# Autodesk Inventor assembly: MIR_HbHand
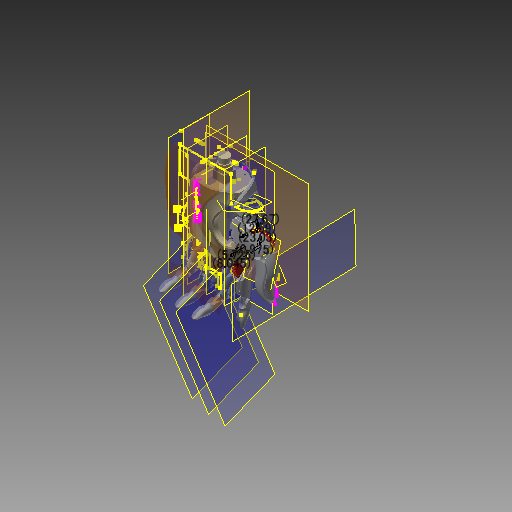
[picture p0: Inventor's stored thumbnail of the model, 512x512]
Saved by Autodesk Inventor 2017 (Build 210142000, 142)
## iProperties
Part Number: MIR_HbHand
Material: 一般
Document SubType Name: Assembly
Designer: sktom
Author: sktom
## Documents named in this file (23)
- D:\OneDrive\CAD\MAJ\hackberry\HACKberry-hardware\3D_69%inlength\Inventor\HbHandForChild\MIR_HbHand.iam
- D:\OneDrive\CAD\MAJ\hackberry\HACKberry-hardware\3D_69%inlength\Inventor\HbHandForChild\MIR_HbPalmBase03ForChild.ipt
- D:\OneDrive\CAD\MAJ\hackberry\HACKberry-hardware\3D_69%inlength\Inventor\HbHandForChild\MIR_bearing_683.ipt
- D:\OneDrive\CAD\MAJ\hackberry\HACKberry-hardware\3D_69%inlength\Inventor\HbHandForChild\HbthumbU02ForChild\MIR_HbthumbU02ForChild.iam
- D:\OneDrive\CAD\MAJ\hackberry\HACKberry-hardware\3D_69%inlength\Inventor\HbHandForChild\HbServoHK282A\MIR_Servo_HK282A_Hone.ipt
- D:\OneDrive\CAD\MAJ\hackberry\HACKberry-hardware\3D_69%inlength\Inventor\HbHandForChild\HbIndexFinger01ForChild\MIR_HbIndexFinger01ForChild.iam
- D:\OneDrive\CAD\MAJ\hackberry\HACKberry-hardware\3D_69%inlength\Inventor\HbHandForChild\HbFinger01ForChild\MIR_HbFinger01ForChild.iam
- D:\OneDrive\CAD\MAJ\hackberry\HACKberry-hardware\3D_69%inlength\Inventor\HbHandForChild\MIR_HbRing-LittleCouplerLink01ForChild.ipt
- D:\OneDrive\CAD\MAJ\hackberry\HACKberry-hardware\3D_69%inlength\Inventor\HbHandForChild\MIR_HbMiddle-RingCouplerLink01ForChild.ipt
- D:\OneDrive\CAD\MAJ\hackberry\HACKberry-hardware\3D_69%inlength\Inventor\HbHandForChild\servo\MIR_Tower Pro 9g Micro Servo SG90.iam
- D:\OneDrive\CAD\MAJ\hackberry\HACKberry-hardware\3D_69%inlength\Inventor\HbHandForChild\MIR_DummyASV-15MG.ipt
- D:\OneDrive\CAD\MAJ\hackberry\HACKberry-hardware\3D_69%inlength\Inventor\HbHandForChild\MIR_HbFingerMainCouplerLink01ForChild.ipt
- D:\OneDrive\CAD\MAJ\hackberry\HACKberry-hardware\3D_69%inlength\Inventor\HbHandForChild\MIR_DummyASV-15MGSingleHorn01.ipt
- D:\OneDrive\CAD\MAJ\hackberry\HACKberry-hardware\3D_69%inlength\Inventor\HbHandForChild\MIR_HbBackCover02ForChild.ipt
- D:\OneDrive\CAD\MAJ\hackberry\HACKberry-hardware\3D_69%inlength\Inventor\HbHandForChild\MIR_Spur Gear (16 teeth).ipt
- D:\OneDrive\CAD\MAJ\hackberry\HACKberry-hardware\3D_69%inlength\Inventor\HbHandForChild\MIR_spacer_2_3_l3.5.ipt
- D:\OneDrive\CAD\MAJ\hackberry\HACKberry-hardware\3D_69%inlength\Inventor\HbHandForChild\MIR_HbServoCover.ipt
- D:\OneDrive\CAD\MAJ\hackberry\HACKberry-hardware\3D_69%inlength\Inventor\HbHandForChild\MIR_HbShaftStopperB04ForChild.ipt
- D:\OneDrive\CAD\MAJ\hackberry\HACKberry-hardware\3D_69%inlength\Inventor\HbHandForChild\MIR_HbShaftStopperA04ForChild.ipt
- D:\OneDrive\CAD\MAJ\hackberry\HACKberry-hardware\3D_69%inlength\Inventor\HbHandForChild\MIR_shaft_phi1.5_l10.ipt
- D:\OneDrive\CAD\MAJ\hackberry\HACKberry-hardware\3D_69%inlength\Inventor\HbHandForChild\MIR_bolt_M2L6.ipt
- D:\OneDrive\CAD\MAJ\hackberry\HACKberry-hardware\3D_69%inlength\Inventor\HbHandForChild\HbCircuit\MIR_HbCircuit.iam
- D:\OneDrive\CAD\MAJ\hackberry\HACKberry-hardware\3D_69%inlength\Inventor\HbHandForChild\HbSwitch\MIR_HbPowerLever05.ipt
## Components (39 placed, 22 different names)
1. MIR_HbPalmBase03ForChild:1 — 挿入:1, 挿入:5, 挿入:4, 挿入:6, 挿入:8, 挿入:7, 挿入:10, 挿入:9, 挿入:12, 挿入:11, 挿入:16, 挿入:15, メイト:3, メイト:2, 挿入:23, 挿入:22, 挿入:32, 挿入:31, 挿入:34, 挿入:33, 挿入:35, 挿入:36, 挿入:37, 挿入:38, 挿入:39, 挿入:41, 挿入:40, 挿入:49
2. MIR_bearing_683:1 — 挿入:1, 挿入:2
3. MIR_HbthumbU02ForChild:1 [sub-assembly] — 挿入:2, 挿入:3
4. MIR_Servo_HK282A_Hone:1 — 挿入:5, 挿入:4, 挿入:3
5. MIR_HbIndexFinger01ForChild:1 [sub-assembly] — 挿入:6
6. MIR_HbFinger01ForChild:1 [sub-assembly] — 挿入:8, 挿入:7, 挿入:30
7. MIR_HbFinger01ForChild:2 [sub-assembly] — 挿入:10, 挿入:9, 挿入:28, 挿入:29
8. MIR_HbFinger01ForChild:3 [sub-assembly] — 挿入:12, 挿入:11, 挿入:19, 挿入:26, 挿入:27
9. MIR_HbRing-LittleCouplerLink01ForChild:1 — フラッシュ:2, 挿入:46, 挿入:47, 円柱状:6, 円柱状:5
10. MIR_HbMiddle-RingCouplerLink01ForChild:1 — フラッシュ:1, 円柱状:3, 円柱状:4
11. MIR_Tower Pro 9g Micro Servo SG90:1 [sub-assembly] — 挿入:16, 挿入:15, 挿入:24
12. MIR_DummyASV-15MG:1 — メイト:3, メイト:2, 挿入:20
13. MIR_HbFingerMainCouplerLink01ForChild:1 — 挿入:19, 挿入:42, 挿入:43
14. MIR_DummyASV-15MGSingleHorn01:1 — 挿入:42, 挿入:20
15. MIR_HbBackCover02ForChild:1 — 挿入:23, 挿入:22
16. MIR_Spur Gear (16 teeth):1 — 挿入:24
17. MIR_spacer_2_3_l3.5:1 — 挿入:26
18. MIR_spacer_2_3_l3.5:2 — 挿入:43, 挿入:48
19. MIR_spacer_2_3_l3.5:3 — フラッシュ:2, 挿入:27, 円柱状:6
20. MIR_spacer_2_3_l3.5:4 — 挿入:28, 円柱状:5
21. MIR_spacer_2_3_l3.5:5 — フラッシュ:1, 挿入:29, 挿入:45, 円柱状:3
22. MIR_spacer_2_3_l3.5:6 — 挿入:30, 挿入:44, 円柱状:4
23. MIR_HbServoCover:1 — 挿入:32, 挿入:31
24. MIR_HbShaftStopperB04ForChild:1 — 挿入:34
25. MIR_HbShaftStopperA04ForChild:1 — 挿入:33
26. MIR_shaft_phi1.5_l10:1 — 挿入:35
27. MIR_shaft_phi1.5_l10:2 — 挿入:36
28. MIR_shaft_phi1.5_l10:3 — 挿入:37
29. MIR_shaft_phi1.5_l10:4 — 挿入:38
30. MIR_shaft_phi1.5_l10:5 — 挿入:39
31. MIR_shaft_phi1.5_l10:6 — 挿入:41
32. MIR_shaft_phi1.5_l10:7 — 挿入:40
33. MIR_bolt_M2L6:1 — 挿入:44
34. MIR_bolt_M2L6:2 — 挿入:45
35. MIR_bolt_M2L6:3 — 挿入:46
36. MIR_bolt_M2L6:4 — 挿入:47
37. MIR_bolt_M2L6:5 — 挿入:48
38. MIR_HbCircuit:1 [sub-assembly] — 挿入:49, メイト:6, メイト:5, メイト:4
39. MIR_HbPowerLever05:1 — メイト:6, メイト:5, メイト:4
## Relationships (54: Insert 43, Mate 5, CylindricalJoint 4, Flush 2)
- 挿入:1 [Insert]: MIR_HbPalmBase03ForChild:1 ↔ MIR_bearing_683:1
- 挿入:2 [Insert]: MIR_bearing_683:1 ↔ MIR_HbthumbU02ForChild:1
- 挿入:5 [Insert]: MIR_HbPalmBase03ForChild:1 ↔ MIR_Servo_HK282A_Hone:1
- 挿入:4 [Insert]: MIR_HbPalmBase03ForChild:1 ↔ MIR_Servo_HK282A_Hone:1
- 挿入:3 [Insert]: MIR_HbthumbU02ForChild:1 ↔ MIR_Servo_HK282A_Hone:1
- 挿入:6 [Insert]: MIR_HbPalmBase03ForChild:1 ↔ MIR_HbIndexFinger01ForChild:1
- 挿入:8 [Insert]: MIR_HbPalmBase03ForChild:1 ↔ MIR_HbFinger01ForChild:1
- 挿入:7 [Insert]: MIR_HbPalmBase03ForChild:1 ↔ MIR_HbFinger01ForChild:1
- 挿入:10 [Insert]: MIR_HbPalmBase03ForChild:1 ↔ MIR_HbFinger01ForChild:2
- 挿入:9 [Insert]: MIR_HbPalmBase03ForChild:1 ↔ MIR_HbFinger01ForChild:2
- 挿入:12 [Insert]: MIR_HbPalmBase03ForChild:1 ↔ MIR_HbFinger01ForChild:3
- 挿入:11 [Insert]: MIR_HbPalmBase03ForChild:1 ↔ MIR_HbFinger01ForChild:3
- 挿入:16 [Insert]: MIR_HbPalmBase03ForChild:1 ↔ MIR_Tower Pro 9g Micro Servo SG90:1
- 挿入:15 [Insert]: MIR_HbPalmBase03ForChild:1 ↔ MIR_Tower Pro 9g Micro Servo SG90:1
- メイト:3 [Mate]: MIR_HbPalmBase03ForChild:1 ↔ MIR_DummyASV-15MG:1
- メイト:2 [Mate]: MIR_HbPalmBase03ForChild:1 ↔ MIR_DummyASV-15MG:1
- 挿入:19 [Insert] (0.1 mm): MIR_HbFinger01ForChild:3 ↔ MIR_HbFingerMainCouplerLink01ForChild:1
- 挿入:42 [Insert]: MIR_HbFingerMainCouplerLink01ForChild:1 ↔ MIR_DummyASV-15MGSingleHorn01:1
- 挿入:20 [Insert]: MIR_DummyASV-15MG:1 ↔ MIR_DummyASV-15MGSingleHorn01:1
- 挿入:23 [Insert]: MIR_HbPalmBase03ForChild:1 ↔ MIR_HbBackCover02ForChild:1
- 挿入:22 [Insert]: MIR_HbPalmBase03ForChild:1 ↔ MIR_HbBackCover02ForChild:1
- 挿入:24 [Insert] (0.8 mm): MIR_Tower Pro 9g Micro Servo SG90:1 ↔ MIR_Spur Gear (16 teeth):1
- 挿入:26 [Insert]: MIR_HbFinger01ForChild:3 ↔ MIR_spacer_2_3_l3.5:1
- 挿入:43 [Insert]: MIR_HbFingerMainCouplerLink01ForChild:1 ↔ MIR_spacer_2_3_l3.5:2
- フラッシュ:2 [Flush]: MIR_HbRing-LittleCouplerLink01ForChild:1 ↔ MIR_spacer_2_3_l3.5:3
- 挿入:27 [Insert]: MIR_HbFinger01ForChild:3 ↔ MIR_spacer_2_3_l3.5:3
- 挿入:28 [Insert]: MIR_HbFinger01ForChild:2 ↔ MIR_spacer_2_3_l3.5:4
- フラッシュ:1 [Flush]: MIR_HbMiddle-RingCouplerLink01ForChild:1 ↔ MIR_spacer_2_3_l3.5:5
- 挿入:29 [Insert]: MIR_HbFinger01ForChild:2 ↔ MIR_spacer_2_3_l3.5:5
- 挿入:30 [Insert]: MIR_HbFinger01ForChild:1 ↔ MIR_spacer_2_3_l3.5:6
- 挿入:32 [Insert]: MIR_HbPalmBase03ForChild:1 ↔ MIR_HbServoCover:1
- 挿入:31 [Insert]: MIR_HbPalmBase03ForChild:1 ↔ MIR_HbServoCover:1
- 挿入:34 [Insert]: MIR_HbPalmBase03ForChild:1 ↔ MIR_HbShaftStopperB04ForChild:1
- 挿入:33 [Insert]: MIR_HbPalmBase03ForChild:1 ↔ MIR_HbShaftStopperA04ForChild:1
- 挿入:35 [Insert]: MIR_HbPalmBase03ForChild:1 ↔ MIR_shaft_phi1.5_l10:1
- 挿入:36 [Insert] (0.5 mm): MIR_HbPalmBase03ForChild:1 ↔ MIR_shaft_phi1.5_l10:2
- 挿入:37 [Insert] (0.3 mm): MIR_HbPalmBase03ForChild:1 ↔ MIR_shaft_phi1.5_l10:3
- 挿入:38 [Insert] (0.3 mm): MIR_HbPalmBase03ForChild:1 ↔ MIR_shaft_phi1.5_l10:4
- 挿入:39 [Insert] (0.5 mm): MIR_HbPalmBase03ForChild:1 ↔ MIR_shaft_phi1.5_l10:5
- 挿入:41 [Insert] (0.5 mm): MIR_HbPalmBase03ForChild:1 ↔ MIR_shaft_phi1.5_l10:6
- 挿入:40 [Insert] (0.5 mm): MIR_HbPalmBase03ForChild:1 ↔ MIR_shaft_phi1.5_l10:7
- 挿入:44 [Insert] (0.3 mm): MIR_spacer_2_3_l3.5:6 ↔ MIR_bolt_M2L6:1
- 挿入:45 [Insert] (0.3 mm): MIR_spacer_2_3_l3.5:5 ↔ MIR_bolt_M2L6:2
- 挿入:46 [Insert] (0.3 mm): MIR_HbRing-LittleCouplerLink01ForChild:1 ↔ MIR_bolt_M2L6:3
- 挿入:47 [Insert] (0.3 mm): MIR_HbRing-LittleCouplerLink01ForChild:1 ↔ MIR_bolt_M2L6:4
- 挿入:48 [Insert] (0.3 mm): MIR_spacer_2_3_l3.5:2 ↔ MIR_bolt_M2L6:5
- 挿入:49 [Insert]: MIR_HbPalmBase03ForChild:1 ↔ MIR_HbCircuit:1
- メイト:6 [Mate] (0.5 mm): MIR_HbCircuit:1 ↔ MIR_HbPowerLever05:1
- メイト:5 [Mate] (0.2 mm): MIR_HbCircuit:1 ↔ MIR_HbPowerLever05:1
- メイト:4 [Mate] (0.2 mm): MIR_HbCircuit:1 ↔ MIR_HbPowerLever05:1
- 円柱状:6 [CylindricalJoint]: MIR_HbRing-LittleCouplerLink01ForChild:1 ↔ MIR_spacer_2_3_l3.5:3
- 円柱状:5 [CylindricalJoint]: MIR_HbRing-LittleCouplerLink01ForChild:1 ↔ MIR_spacer_2_3_l3.5:4
- 円柱状:3 [CylindricalJoint]: MIR_HbMiddle-RingCouplerLink01ForChild:1 ↔ MIR_spacer_2_3_l3.5:5
- 円柱状:4 [CylindricalJoint]: MIR_HbMiddle-RingCouplerLink01ForChild:1 ↔ MIR_spacer_2_3_l3.5:6
